# Autodesk Inventor assembly: Assembly1
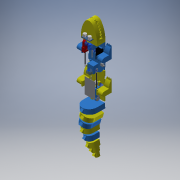
[picture p0: Inventor's stored thumbnail of the model, 180x180]
Saved by Autodesk Inventor 2016 (Build 200138000, 138)
## iProperties
Created: 2017-03-04
Part Number: Assembly1
Document SubType Name: Assembly
Designer: Owner
Author: Owner
## Documents named in this file (37)
- C:\Users\Owner\Documents\Inventor\TSA\2017\Animatronics\Alligator\Alligator\Assembly1.iam
- C:\Users\Owner\Documents\Inventor\TSA\2017\Animatronics\Alligator\Alligator\Frame\Fronthalf.ipt
- C:\Users\Owner\Documents\Inventor\TSA\2017\Animatronics\Alligator\Alligator\Frame\Backhalf.ipt
- C:\Users\Owner\Documents\Inventor\TSA\2017\Animatronics\Alligator\Mock Parts\servo (2).ipt
- C:\Users\Owner\Documents\Inventor\TSA\2017\Animatronics\Alligator\Pistons\Syringe1mL\SyringeBody.ipt
- C:\Users\Owner\Documents\Inventor\TSA\2017\Animatronics\Alligator\Alligator\Skin\Skin1.ipt
- C:\Users\Owner\Documents\Inventor\TSA\2017\Animatronics\Alligator\Pistons\Syringe1mL\SyringEnd.ipt
- C:\Users\Owner\Documents\Inventor\TSA\2017\Animatronics\Alligator\Alligator\Tail\Tail1.ipt
- C:\Users\Owner\Documents\Inventor\TSA\2017\Animatronics\Alligator\Alligator\Tail\Tail2.ipt
- C:\Users\Owner\Documents\Inventor\TSA\2017\Animatronics\Alligator\Alligator\Tail\Tail3.ipt
- C:\Users\Owner\Documents\Inventor\TSA\2017\Animatronics\Alligator\Alligator\Tail\Tail4.ipt
- C:\Users\Owner\Documents\Inventor\TSA\2017\Animatronics\Alligator\Alligator\Tail\Tail5.ipt
- C:\Users\Owner\Documents\Inventor\TSA\2017\Animatronics\Alligator\Alligator\Tail\Tail6.ipt
- C:\Users\Owner\Documents\Inventor\TSA\2017\Animatronics\Alligator\Alligator\Tail\SyringeTailConnector.ipt
- C:\Users\Owner\Documents\Inventor\TSA\2017\Animatronics\Alligator\Alligator\Tail\ConnectingBlockTail.ipt
- C:\Users\Owner\Documents\Inventor\TSA\2017\Animatronics\Alligator\Alligator\Tail\TailConnector2.ipt
- C:\Users\Owner\Documents\Inventor\TSA\2017\Animatronics\Alligator\Pistons\PistonTailV2 - Copy\PistonV2.iam
- C:\Users\Owner\Documents\Inventor\TSA\2017\Animatronics\Alligator\Alligator\Reference\Gear.ipt
- C:\Users\Owner\Documents\Inventor\TSA\2017\Animatronics\Alligator\Pistons\PistonHead\PistonV2.iam
- C:\Users\Owner\Documents\Inventor\TSA\2017\Animatronics\Alligator\Mock Parts\9Volt.ipt
- C:\Users\Owner\Documents\Inventor\TSA\2017\Animatronics\Alligator\Alligator\Frame\StupidPiece.ipt
- C:\Users\Owner\Documents\Inventor\TSA\2017\Animatronics\Alligator\Alligator\Skin\Skin2V2.ipt
- C:\Users\Owner\Documents\Inventor\TSA\2017\Animatronics\Alligator\Alligator\Skin\Skin3.ipt
- C:\Users\Owner\Documents\Inventor\TSA\2017\Animatronics\Alligator\Alligator\Skin\Skin4.ipt
- C:\Users\Owner\Documents\Inventor\TSA\2017\Animatronics\Alligator\Alligator\Frame\ConnectorRodBodies.ipt
- C:\Users\Owner\Documents\Inventor\TSA\2017\Animatronics\Alligator\Alligator\Frame\LargeConnectorBodies.ipt
- C:\Users\Owner\Documents\Inventor\TSA\2017\Animatronics\Alligator\Alligator\Legs\Leg.ipt
- C:\Users\Owner\Documents\Inventor\D3D Crawl\Movement\Idler Bearing.ipt
- C:\Users\Owner\Documents\Inventor\TSA\2017\Animatronics\Alligator\Alligator\Legs\Leg_MIR.ipt
- C:\Users\Owner\Documents\Inventor\TSA\2017\Animatronics\Alligator\Alligator\Frame\HeadFrame.ipt
- C:\Users\Owner\Documents\Inventor\TSA\2017\Animatronics\Alligator\Alligator\Frame\HeadSKin.ipt
- C:\Users\Owner\Documents\Inventor\TSA\2017\Animatronics\Alligator\Alligator\Hinge.ipt
- C:\Users\Owner\Documents\3D Printing\TSA\2017\Alligator\Tail\Toungue.ipt
- C:\Users\Owner\Documents\Inventor\TSA\2017\Animatronics\Alligator\Alligator\Wheel.ipt
- C:\Users\Owner\Documents\Inventor\TSA\2017\Animatronics\Alligator\Mock Parts\uno.ipt
- C:\Users\Owner\Documents\Inventor\TSA\2017\Animatronics\Alligator\Mock Parts\HC-SR04.ipt
- C:\Users\Owner\Documents\Inventor\TSA\2017\Animatronics\Alligator\Mock Parts\Toggle Switch.ipt
## Components (45 placed, 35 different names)
1. Fronthalf:1 — Flush:1, Mate:1, Flush:14, Mate:13, Flush:17, Flush:18, Mate:34, Mate:35, Mate:36, Mate:38, Flush:43, Flush:44, Mate:39, Angle:8, Flush:45, Flush:46, Mate:45, Flush:48, Flush:66, Mate:72, Flush:68, Flush:69, Flush:71, Flush:78, Mate:108, Flush:88
2. Backhalf:1 — Flush:1, Mate:1, Mate:17, Flush:22, Mate:43, Mate:44, Mate:48, Flush:52, Mate:51, Mate:52, Flush:56, Flush:63, Mate:68, Flush:64, Mate:70, Flush:65, Flush:68, Flush:70, Flush:72, Mate:73
3. SyringeBody:1 — Flush:14
4. Skin1:1 — Mate:13, Flush:17, Flush:18, Mate:71, Mate:75, Flush:74, Mate:78, Mate:93, Mate:99, Mate:102, Mate:106
5. SyringeBody:2 — Mate:17, Flush:22, Mate:53
6. servo (2):6 — Mate:34, Mate:35, Flush:71
7. PistonV2:1 [sub-assembly] — Mate:36, Mate:38, Flush:43, Flush:44
8. Gear:1 — Mate:39, Mate:41, Mate:42
9. servo (2):7 — Mate:41, Mate:42, Angle:8, Flush:45, Flush:46
10. PistonV2:2 [sub-assembly] — Flush:51, Mate:48, Flush:52, Flush:87
11. servo (2):8 — Mate:43, Mate:44, Flush:51, Flush:70, Flush:84
12. 9Volt:1 — Mate:45, Flush:48
13. StupidPiece:1 — Mate:51, Mate:52, Angle:9, Mate:59
14. SyringeTailConnector:1 — Mate:54, Flush:55, Angle:9, Mate:55, Mate:56
15. TailConnector2:1 — Mate:55, Mate:56, Mate:62
16. SyringEnd:1 — Mate:53, Mate:54, Flush:55
17. Tail1:1 — Mate:59, Flush:56, Mate:60, Mate:61, Flush:57, Mate:67, Flush:62
18. Tail2:1 — Flush:58, Mate:66, Mate:67, Flush:62
19. Tail3:1 — Flush:58, Flush:59, Mate:65, Mate:66
20. Tail4:1 — Flush:59, Flush:60, Mate:64, Mate:65
21. Tail5:1 — Flush:60, Flush:61, Mate:63, Mate:64
22. Tail6:1 — Flush:61, Mate:63
23. ConnectingBlockTail:2 — Mate:60, Mate:61, Flush:57, Mate:62
24. Skin2V2:1 — Mate:71, Flush:66, Mate:72, Flush:73, Mate:74, Mate:79
25. Skin3:1 — Mate:69, Mate:70, Flush:65, Flush:75, Flush:76, Flush:77, Mate:84, Mate:85
26. Skin4:1 — Flush:63, Mate:68, Flush:64, Mate:69, Mate:82, Mate:83
27. LargeConnectorBodies:1 — Flush:69, Flush:72
28. ConnectorRodBodies:1 — Mate:73
29. Idler Bearing:3 — Mate:76, Mate:77
30. Idler Bearing:4 — Mate:80, Mate:81
31. Idler Bearing:5 — Mate:86, Mate:89
32. Idler Bearing:6 — Mate:87, Mate:88
33. Leg:1 — Flush:73, Mate:74, Mate:75, Mate:76, Mate:77
34. Leg_MIR:1 — Flush:74, Mate:78, Mate:79, Mate:80, Mate:81
35. Leg_MIR:2 — Flush:75, Flush:76, Mate:82, Mate:83, Mate:87, Mate:88
36. Leg:2 — Flush:77, Mate:84, Mate:85, Mate:86, Mate:89
37. HeadFrame:1 — Flush:78, Mate:99, Flush:83, Mate:105, Flush:85
38. Hinge:1 — Mate:93, Flush:86
39. HeadSKin:1 — Mate:105, Flush:85, Mate:106, Flush:86, Mate:107
40. Toungue:1 — Flush:83
41. SyringEnd:2 — Mate:102
42. Wheel:1 — Flush:84
43. uno:1 — Flush:87
44. HC-SR04:1 — Mate:107
45. Toggle Switch:1 — Mate:108, Flush:88
## Relationships (101: Mate 58, Flush 41, Angle 2)
- Flush:1: Fronthalf:1 ↔ Backhalf:1
- Mate:1: Fronthalf:1 ↔ Backhalf:1
- Flush:14: Fronthalf:1 ↔ SyringeBody:1
- Mate:13: Fronthalf:1 ↔ Skin1:1
- Flush:17: Fronthalf:1 ↔ Skin1:1
- Flush:18: Fronthalf:1 ↔ Skin1:1
- Mate:17: Backhalf:1 ↔ SyringeBody:2
- Flush:22 (10 mm): Backhalf:1 ↔ SyringeBody:2
- Mate:34: Fronthalf:1 ↔ servo (2):6
- Mate:35: Fronthalf:1 ↔ servo (2):6
- Mate:36: Fronthalf:1 ↔ PistonV2:1
- Mate:38 (0.508 mm): Fronthalf:1 ↔ PistonV2:1
- Flush:43: Fronthalf:1 ↔ PistonV2:1
- Flush:44: Fronthalf:1 ↔ PistonV2:1
- Mate:39: Fronthalf:1 ↔ Gear:1
- Mate:41: Gear:1 ↔ servo (2):7
- Mate:42: Gear:1 ↔ servo (2):7
- Angle:8 (0 deg): Fronthalf:1 ↔ servo (2):7
- Flush:45: Fronthalf:1 ↔ servo (2):7
- Flush:46: Fronthalf:1 ↔ servo (2):7
- Mate:43: Backhalf:1 ↔ servo (2):8
- Mate:44: Backhalf:1 ↔ servo (2):8
- Mate:45: Fronthalf:1 ↔ 9Volt:1
- Flush:48 (-4.45 mm): Fronthalf:1 ↔ 9Volt:1
- Flush:51: PistonV2:2 ↔ servo (2):8
- Mate:48: Backhalf:1 ↔ PistonV2:2
- Flush:52: Backhalf:1 ↔ PistonV2:2
- Mate:51: Backhalf:1 ↔ StupidPiece:1
- Mate:52: Backhalf:1 ↔ StupidPiece:1
- Mate:53: SyringeBody:2 ↔ SyringEnd:1
- Mate:54: SyringeTailConnector:1 ↔ SyringEnd:1
- Flush:55 (0.5 mm): SyringeTailConnector:1 ↔ SyringEnd:1
- Angle:9 (0 deg): StupidPiece:1 ↔ SyringeTailConnector:1
- Mate:55: SyringeTailConnector:1 ↔ TailConnector2:1
- Mate:56: SyringeTailConnector:1 ↔ TailConnector2:1
- Mate:59: StupidPiece:1 ↔ Tail1:1
- Flush:56: Backhalf:1 ↔ Tail1:1
- Mate:60: Tail1:1 ↔ ConnectingBlockTail:2
- Mate:61: Tail1:1 ↔ ConnectingBlockTail:2
- Flush:57: Tail1:1 ↔ ConnectingBlockTail:2
- Mate:62: TailConnector2:1 ↔ ConnectingBlockTail:2
- Flush:58: Tail2:1 ↔ Tail3:1
- Flush:59: Tail3:1 ↔ Tail4:1
- Flush:60: Tail4:1 ↔ Tail5:1
- Flush:61: Tail5:1 ↔ Tail6:1
- Mate:63: Tail5:1 ↔ Tail6:1
- Mate:64: Tail4:1 ↔ Tail5:1
- Mate:65: Tail3:1 ↔ Tail4:1
- Mate:66: Tail2:1 ↔ Tail3:1
- Mate:67: Tail1:1 ↔ Tail2:1
- Flush:62: Tail1:1 ↔ Tail2:1
- Flush:63: Backhalf:1 ↔ Skin4:1
- Mate:68: Backhalf:1 ↔ Skin4:1
- Flush:64: Backhalf:1 ↔ Skin4:1
- Mate:69: Skin3:1 ↔ Skin4:1
- Mate:70: Backhalf:1 ↔ Skin3:1
- Flush:65: Backhalf:1 ↔ Skin3:1
- Mate:71: Skin1:1 ↔ Skin2V2:1
- Flush:66: Fronthalf:1 ↔ Skin2V2:1
- Mate:72: Fronthalf:1 ↔ Skin2V2:1
- Flush:68: Fronthalf:1 ↔ Backhalf:1
- Flush:69: Fronthalf:1 ↔ LargeConnectorBodies:1
- Flush:70: Backhalf:1 ↔ servo (2):8
- Flush:71: Fronthalf:1 ↔ servo (2):6
- Flush:72: Backhalf:1 ↔ LargeConnectorBodies:1
- Mate:73: Backhalf:1 ↔ ConnectorRodBodies:1
- Flush:73: Skin2V2:1 ↔ Leg:1
- Mate:74 (0.25 mm): Skin2V2:1 ↔ Leg:1
- Mate:75 (0.25 mm): Skin1:1 ↔ Leg:1
- Mate:76: Idler Bearing:3 ↔ Leg:1
- Mate:77 (0.5 mm): Idler Bearing:3 ↔ Leg:1
- Flush:74: Skin1:1 ↔ Leg_MIR:1
- Mate:78 (0.25 mm): Skin1:1 ↔ Leg_MIR:1
- Mate:79 (0.25 mm): Skin2V2:1 ↔ Leg_MIR:1
- Mate:80: Idler Bearing:4 ↔ Leg_MIR:1
- Mate:81 (0.5 mm): Idler Bearing:4 ↔ Leg_MIR:1
- Flush:75: Skin3:1 ↔ Leg_MIR:2
- Flush:76: Skin3:1 ↔ Leg_MIR:2
- Mate:82 (0.25 mm): Skin4:1 ↔ Leg_MIR:2
- Mate:83 (0.25 mm): Skin4:1 ↔ Leg_MIR:2
- Flush:77: Skin3:1 ↔ Leg:2
- Mate:84 (0.25 mm): Skin3:1 ↔ Leg:2
- Mate:85 (0.25 mm): Skin3:1 ↔ Leg:2
- Mate:86: Idler Bearing:5 ↔ Leg:2
- Mate:87: Idler Bearing:6 ↔ Leg_MIR:2
- Mate:88 (0.5 mm): Idler Bearing:6 ↔ Leg_MIR:2
- Mate:89 (0.5 mm): Idler Bearing:5 ↔ Leg:2
- Flush:78: Fronthalf:1 ↔ HeadFrame:1
- Mate:93: Skin1:1 ↔ Hinge:1
- Mate:99: Skin1:1 ↔ HeadFrame:1
- Flush:83: HeadFrame:1 ↔ Toungue:1
- Mate:102: Skin1:1 ↔ SyringEnd:2
- Flush:84: servo (2):8 ↔ Wheel:1
- Mate:105: HeadFrame:1 ↔ HeadSKin:1
- Flush:85: HeadFrame:1 ↔ HeadSKin:1
- Mate:106: Skin1:1 ↔ HeadSKin:1
- Flush:86: Hinge:1 ↔ HeadSKin:1
- Flush:87: PistonV2:2 ↔ uno:1
- Mate:107: HeadSKin:1 ↔ HC-SR04:1
- Mate:108: Fronthalf:1 ↔ Toggle Switch:1
- Flush:88: Fronthalf:1 ↔ Toggle Switch:1
